# Autodesk Inventor assembly: base short wall
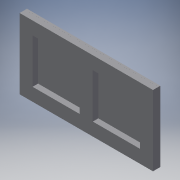
[picture p0: Inventor's stored thumbnail of the model, 180x180]
Saved by Autodesk Inventor 2017 (Build 210142000, 142)
## iProperties
Created: 2019-05-05
Part Number: base short wall
Document SubType Name: Assembly
Designer: Roman
Author: Roman
## Documents named in this file (4)
- C:\Users\Roman\Documents\CAD\tegu rev2\base\short wall\base short wall.iam
- C:\Users\Roman\Documents\CAD\tegu rev2\base\short wall\base short wall h bar.ipt
- C:\Users\Roman\Documents\CAD\tegu rev2\base\short wall\base short wall v bar.ipt
- C:\Users\Roman\Documents\CAD\tegu rev2\base\short wall\base short wall back.ipt
## Components (6 placed, 3 different names)
1. base short wall h bar:1 — Mate:1, Flush:1, Flush:2
2. base short wall h bar:2 — Flush:3, Mate:2, Flush:4, Mate:3, Mate:4, Flush:5
3. base short wall back:1 — Mate:3, Mate:4, Flush:5, Flush:6
4. base short wall v bar:1 — Mate:1, Flush:1, Flush:2, Flush:3, Mate:2, Flush:4
5. base short wall v bar:2
6. base short wall v bar:3 — Flush:6
## Component patterns: (3 elements, first: base short wall v bar:1)
## Relationships (10: Flush 6, Mate 4)
- Mate:1: base short wall h bar:1 ↔ base short wall v bar:1
- Flush:1: base short wall h bar:1 ↔ base short wall v bar:1
- Flush:2: base short wall h bar:1 ↔ base short wall v bar:1
- Flush:3: base short wall h bar:2 ↔ base short wall v bar:1
- Mate:2: base short wall h bar:2 ↔ base short wall v bar:1
- Flush:4: base short wall h bar:2 ↔ base short wall v bar:1
- Mate:3: base short wall h bar:2 ↔ base short wall back:1
- Mate:4: base short wall h bar:2 ↔ base short wall back:1
- Flush:5: base short wall h bar:2 ↔ base short wall back:1
- Flush:6: base short wall back:1 ↔ base short wall v bar:3
